# Autodesk Inventor assembly: nano cam assem
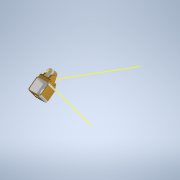
[picture p0: Inventor's stored thumbnail of the model, 180x180]
Saved by Autodesk Inventor 2020 (Build 240168000, 168)
## iProperties
Created: 2022-06-24
Part Number: nano cam assem
Document SubType Name: Assembly
Designer: Steven
Author: Steven
## Documents named in this file (3)
- Y:\FPV drone stuff\0 Street League\Frames\PB-Kauri-X\3D prints\35 mm canopy\work in progress prints\session mounts\nano cam assem.iam
- Y:\FPV drone stuff\0 Street League\Frames\PB-Kauri-X\3D prints\35 mm canopy\work in progress prints\session mounts\V1 session mount.ipt
- Y:\FPV drone stuff\0 Street League\Frames\PB-Kauri-X\3D prints\35 mm canopy\work in progress prints\Camera mounts\predator nano\45 deg predator nano mount.ipt
## Components (2 placed, 2 different names)
1. V1 session mount:1 — Flush:1, Mate:1, Mate:2
2. 45 deg predator nano mount:1 — Flush:1, Mate:1, Mate:2
## Relationships (3: Mate 2, Flush 1)
- Flush:1 (6.15 mm): V1 session mount:1 ↔ 45 deg predator nano mount:1
- Mate:1: V1 session mount:1 ↔ 45 deg predator nano mount:1
- Mate:2: V1 session mount:1 ↔ 45 deg predator nano mount:1
